# Autodesk Inventor assembly: Puzzle Cube
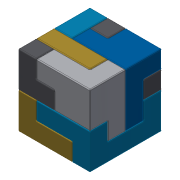
[picture p0: Inventor's stored thumbnail of the model, 180x180]
Saved by Autodesk Inventor 2014 (Build 180170000, 170)
## iProperties
Created: 2013-06-22
Part Number: Puzzle Cube
Document SubType Name: Assembly
Designer: ACooper
Mass: 19.2957 g
Surface Area: 387.084 cm^2
Volume: 19.2957 cm^3
Density: 1 g/cm^3
VLDS_Profile: Default Assembly
VLDS_TimeStamp: 2013-08-25
VLDS_FailCnt: 9
VLDS_AcceptCnt: 0
Author: ACooper
## Documents named in this file (11)
- C:\Ascent ADSK Courses\Inventor 2014 Introduction to Modeling\Puzzle Cube\Puzzle Cube.iam
- C:\Ascent ADSK Courses\Inventor 2014 Introduction to Modeling\Puzzle Cube\Cube Master.ipt
- C:\Ascent ADSK Courses\Inventor 2014 Introduction to Modeling\Puzzle Cube\Piece 1.ipt
- C:\Ascent ADSK Courses\Inventor 2014 Introduction to Modeling\Puzzle Cube\Piece 2.ipt
- C:\Ascent ADSK Courses\Inventor 2014 Introduction to Modeling\Puzzle Cube\Piece 3.ipt
- C:\Ascent ADSK Courses\Inventor 2014 Introduction to Modeling\Puzzle Cube\Piece 4.ipt
- C:\Ascent ADSK Courses\Inventor 2014 Introduction to Modeling\Puzzle Cube\Piece 5.ipt
- C:\Ascent ADSK Courses\Inventor 2014 Introduction to Modeling\Puzzle Cube\Piece 6.ipt
- C:\Ascent ADSK Courses\Inventor 2014 Introduction to Modeling\Puzzle Cube\Piece 7.ipt
- C:\Ascent ADSK Courses\Inventor 2014 Introduction to Modeling\Puzzle Cube\Piece 8.ipt
- C:\Ascent ADSK Courses\Inventor 2014 Introduction to Modeling\Puzzle Cube\Piece 9.ipt
## Components (10 placed, 10 different names)
1. Cube Master:1 — Flush:1, Flush:2, Flush:3, Flush:4, Flush:5, Flush:6, Flush:7, Flush:8, Flush:9, Flush:10, Flush:11, Flush:12, Flush:13, Flush:14, Flush:15, Flush:16, Flush:17, Flush:18, Flush:19, Flush:20, Flush:21, Flush:22, Flush:23, Flush:24, Flush:25, Flush:26, Flush:27
2. Piece 1:1 — Flush:1, Flush:2, Flush:3
3. Piece 2:1 — Flush:4, Flush:5, Flush:6
4. Piece 3:1 — Flush:7, Flush:8, Flush:9
5. Piece 4:1 — Flush:10, Flush:11, Flush:12
6. Piece 5:1 — Flush:13, Flush:14, Flush:15
7. Piece 6:1 — Flush:16, Flush:17, Flush:18
8. Piece 7:1 — Flush:19, Flush:20, Flush:21
9. Piece 8:1 — Flush:22, Flush:23, Flush:24
10. Piece 9:1 — Flush:25, Flush:26, Flush:27
## Relationships (27: Flush 27)
- Flush:1: Cube Master:1 ↔ Piece 1:1
- Flush:2: Cube Master:1 ↔ Piece 1:1
- Flush:3: Cube Master:1 ↔ Piece 1:1
- Flush:4: Cube Master:1 ↔ Piece 2:1
- Flush:5: Cube Master:1 ↔ Piece 2:1
- Flush:6: Cube Master:1 ↔ Piece 2:1
- Flush:7: Cube Master:1 ↔ Piece 3:1
- Flush:8: Cube Master:1 ↔ Piece 3:1
- Flush:9: Cube Master:1 ↔ Piece 3:1
- Flush:10: Cube Master:1 ↔ Piece 4:1
- Flush:11: Cube Master:1 ↔ Piece 4:1
- Flush:12: Cube Master:1 ↔ Piece 4:1
- Flush:13: Cube Master:1 ↔ Piece 5:1
- Flush:14: Cube Master:1 ↔ Piece 5:1
- Flush:15: Cube Master:1 ↔ Piece 5:1
- Flush:16: Cube Master:1 ↔ Piece 6:1
- Flush:17: Cube Master:1 ↔ Piece 6:1
- Flush:18: Cube Master:1 ↔ Piece 6:1
- Flush:19: Cube Master:1 ↔ Piece 7:1
- Flush:20: Cube Master:1 ↔ Piece 7:1
- Flush:21: Cube Master:1 ↔ Piece 7:1
- Flush:22: Cube Master:1 ↔ Piece 8:1
- Flush:23: Cube Master:1 ↔ Piece 8:1
- Flush:24: Cube Master:1 ↔ Piece 8:1
- Flush:25: Cube Master:1 ↔ Piece 9:1
- Flush:26: Cube Master:1 ↔ Piece 9:1
- Flush:27: Cube Master:1 ↔ Piece 9:1
